# Autodesk Inventor assembly: Switch on T nut with holder
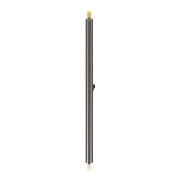
[picture p0: Inventor's stored thumbnail of the model, 180x180]
Saved by Autodesk Inventor 2018 (Build 220112000, 112)
## iProperties
Created: 2018-11-29
Part Number: Switch on T nut with holder
Document SubType Name: Assembly
Designer: ball
Author: ball
## Documents named in this file (5)
- C:\FTC\FTC8863CAD\2018Robot\Switch on T nut with holder.iam
- C:\FTC\FTC8863CAD\Actobotics\585 parts\585718.ipt
- C:\FTC\FTC8863CAD\Actobotics\605 parts\605630.ipt
- C:\FTC\FTC8863CAD\Actobotics\565 parts\565150.ipt
- C:\FTC\FTC8863CAD\2018Robot\Switch on T nut holder.ipt
## Components (4 placed, 4 different names)
1. 585718:1 — Mate:1, Flush:1, Mate:2, Flush:2, Flush:3
2. 605630:1 — Mate:1, Flush:1, Flush:2
3. 565150:1 — Mate:2, Flush:3, Flush:4, Flush:5
4. Switch on T nut holder:1 — Flush:4, Flush:5
## Relationships (7: Flush 5, Mate 2)
- Mate:1 (5.08 mm): 585718:1 ↔ 605630:1
- Flush:1 (-2.54 mm): 585718:1 ↔ 605630:1
- Mate:2: 585718:1 ↔ 565150:1
- Flush:2 (10.16 mm): 585718:1 ↔ 605630:1
- Flush:3: 585718:1 ↔ 565150:1
- Flush:4: 565150:1 ↔ Switch on T nut holder:1
- Flush:5: 565150:1 ↔ Switch on T nut holder:1
